# Autodesk Inventor assembly: デフォルト指アセンブリ
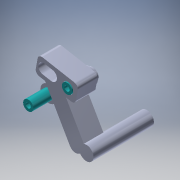
[picture p0: Inventor's stored thumbnail of the model, 180x180]
Saved by Autodesk Inventor 2018 (Build 220112000, 112)
## iProperties
Created: 2018-12-25
Part Number: デフォルト指アセンブリ
Material: 一般
Document SubType Name: Assembly
Designer: lowyu
Author: lowyu
## Documents named in this file (5)
- C:\Users\lowyu\Desktop\HAND\シャッターハンド\卒論\デフォルト指アセンブリ.iam
- C:\Users\lowyu\Desktop\HAND\シャッターハンド\指v5.ipt
- C:\Users\lowyu\Desktop\HAND\シャッターハンド\座金.ipt
- C:\Users\lowyu\Desktop\HAND\シャッターハンド\CBSA3-5 極低頭六角穴付ボルト.ipt
- C:\Users\lowyu\Desktop\HAND\シャッターハンド\内側　支柱.ipt
## Components (7 placed, 4 different names)
1. 指v5:1 — メイト:1, フラッシュ:1, メイト:2, メイト:10
2. 座金:1 — メイト:2, メイト:3, メイト:4, メイト:5
3. CBSA3-5 極低頭六角穴付ボルト:1 — メイト:4, メイト:5
4. CBSA3-5 極低頭六角穴付ボルト:2 — メイト:8, メイト:9
5. 座金:2 — メイト:6, メイト:7, メイト:8, メイト:10
6. 内側　支柱:1 — メイト:6, メイト:7, メイト:9
7. 内側　支柱:2 — メイト:1, フラッシュ:1, メイト:3
## Relationships (11: Mate 10, Flush 1)
- メイト:1 [Mate]: 指v5:1 ↔ 内側　支柱:2
- フラッシュ:1 [Flush]: 指v5:1 ↔ 内側　支柱:2
- メイト:2 [Mate]: 指v5:1 ↔ 座金:1
- メイト:3 [Mate]: 座金:1 ↔ 内側　支柱:2
- メイト:4 [Mate]: 座金:1 ↔ CBSA3-5 極低頭六角穴付ボルト:1
- メイト:5 [Mate]: 座金:1 ↔ CBSA3-5 極低頭六角穴付ボルト:1
- メイト:6 [Mate]: 座金:2 ↔ 内側　支柱:1
- メイト:7 [Mate]: 座金:2 ↔ 内側　支柱:1
- メイト:8 [Mate]: CBSA3-5 極低頭六角穴付ボルト:2 ↔ 座金:2
- メイト:9 [Mate]: CBSA3-5 極低頭六角穴付ボルト:2 ↔ 内側　支柱:1
- メイト:10 [Mate]: 指v5:1 ↔ 座金:2
